# Autodesk Inventor assembly: Ensamblaje5
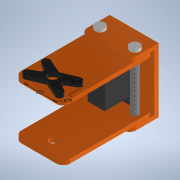
[picture p0: Inventor's stored thumbnail of the model, 180x180]
Saved by Autodesk Inventor 2021 (Build 250183000, 183)
## iProperties
Created: 2021-04-03
Part Number: Ensamblaje5
Document SubType Name: Assembly
Designer: diego
Author: diego
## Documents named in this file (7)
- C:\Users\diego\Desktop\Diego\Utadeo 2021-1\Robotica Industrial\Corte 2\Solido planos\Ensamblaje5.iam
- C:\Users\diego\Desktop\Diego\Utadeo 2021-1\Robotica Industrial\Corte 2\Solido planos\5.ipt
- C:\Users\diego\Desktop\Diego\Utadeo 2021-1\Robotica Industrial\Corte 2\Solido planos\Extension2.ipt
- C:\Users\diego\Desktop\Diego\Utadeo 2021-1\Robotica Industrial\Corte 2\Solido planos\6.ipt
- C:\Users\diego\Desktop\Diego\Utadeo 2021-1\Robotica Industrial\Corte 2\Solido planos\Tornillo_Corto.ipt
- C:\Users\diego\Desktop\Diego\Utadeo 2021-1\Robotica Industrial\Corte 2\Gripper\MG90S Servo Motor.ipt
- C:\Users\diego\Desktop\Diego\Utadeo 2021-1\Robotica Industrial\Corte 2\Solido planos\8_1.ipt
## Components (7 placed, 6 different names)
1. 5:1 — Coincidencia:1, Coincidencia:2, De rotación:1, Rígido:1
2. Extension2:1 — Coincidencia:1, Coincidencia:2
3. 6:1 — Rígido:2
4. Tornillo_Corto:1
5. Tornillo_Corto:2
6. MG90S Servo Motor:1
7. 8_1:1 — De rotación:1, Rígido:1, Rígido:2
## Relationships (5: Mate 2, WeldJoint 2, RevoluteJoint 1)
- Coincidencia:1 [Mate]: 5:1 ↔ Extension2:1
- Coincidencia:2 [Mate]: 5:1 ↔ Extension2:1
- De rotación:1 [RevoluteJoint]: 5:1 ↔ 8_1:1
- Rígido:1 [WeldJoint]: 5:1 ↔ 8_1:1
- Rígido:2 [WeldJoint]: 6:1 ↔ 8_1:1
